# Autodesk Inventor assembly: Assembly
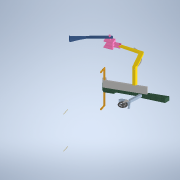
[picture p0: Inventor's stored thumbnail of the model, 180x180]
Saved by Autodesk Inventor 2021 (Build 250183000, 183)
## iProperties
Created: 2021-05-09
Part Number: Assembly
Document SubType Name: Assembly
Designer: Alsayaary
Author: Abdulrahman
## Documents named in this file (11)
- C:\Users\ocon0143\OneDrive - Flinders\Advn Mech Design Shared\6_Development\2_Design\inventor\securing_mechanism\Assembly.iam
- C:\Users\ocon0143\OneDrive - Flinders\Advn Mech Design Shared\6_Development\2_Design\inventor\securing_mechanism\grip - C1-1.ipt
- C:\Users\ocon0143\OneDrive - Flinders\Advn Mech Design Shared\6_Development\2_Design\inventor\securing_mechanism\grip - C2-1.ipt
- C:\Users\ocon0143\OneDrive - Flinders\Advn Mech Design Shared\6_Development\2_Design\inventor\securing_mechanism\grip - C4-1.ipt
- C:\Users\ocon0143\OneDrive - Flinders\Advn Mech Design Shared\6_Development\2_Design\inventor\securing_mechanism\pin-1.ipt
- C:\Users\ocon0143\OneDrive - Flinders\Advn Mech Design Shared\6_Development\2_Design\inventor\securing_mechanism\sweep.ipt
- C:\Users\ocon0143\OneDrive - Flinders\Advn Mech Design Shared\6_Development\2_Design\inventor\securing_mechanism\wheel2.ipt
- C:\Users\ocon0143\OneDrive - Flinders\Advn Mech Design Shared\6_Development\2_Design\inventor\securing_mechanism\grip - Copy1-1.ipt
- C:\Users\ocon0143\OneDrive - Flinders\Advn Mech Design Shared\6_Development\2_Design\inventor\securing_mechanism\handle.ipt
- C:\Users\ocon0143\OneDrive - Flinders\Advn Mech Design Shared\6_Development\2_Design\inventor\securing_mechanism\grip_N_fix.ipt
- C:\Users\ocon0143\OneDrive - Flinders\Advn Mech Design Shared\6_Development\2_Design\inventor\securing_mechanism\secure_wheel_bar.ipt
## Components (10 placed, 10 different names)
1. grip - C1-1:1 — Mate:1, Mate:2, Flush:1, Mate:3, Flush:2, Mate:4, Mate:5, Mate:7, Mate:8, Flush:3, Mate:14, Transitional:1, Mate:23
2. grip - C2-1:1 — Mate:5, Mate:7, Mate:8, Flush:3, Mate:16, Mate:17, Mate:19, Mate:22
3. grip - C4-1:1 — Mate:3, Flush:2, Mate:4, Mate:15
4. sweep:1 — Mate:9, Mate:10, Transitional:1
5. wheel2:1 — Mate:15, Angle:3
6. pin-1:2 — Mate:16, Mate:18
7. grip - Copy1-1:1 — Mate:17, Mate:18, Mate:19, Mate:20, Mate:21
8. handle:1 — Mate:20, Mate:21
9. grip_N_fix:1 — Mate:23
10. secure_wheel_bar:1 — Mate:22
## Relationships (30: Mate 21, Flush 4, Angle 3, Symmetry 1, Transitional 1)
- Mate:1: grip - C1-1:1
- Mate:2: grip - C1-1:1
- Flush:1: grip - C1-1:1
- Mate:3: grip - C1-1:1 ↔ grip - C4-1:1
- Flush:2 (6.27 mm): grip - C1-1:1 ↔ grip - C4-1:1
- Mate:4 (231.798 mm): grip - C1-1:1 ↔ grip - C4-1:1
- Mate:5: grip - C1-1:1 ↔ grip - C2-1:1
- Mate:7: grip - C1-1:1 ↔ grip - C2-1:1
- Mate:8 (313.691 mm): grip - C1-1:1 ↔ grip - C2-1:1
- Flush:3: grip - C1-1:1 ↔ grip - C2-1:1
- Mate:9: sweep:1
- Mate:10: sweep:1
- Mate:11
- Angle:1 (0 deg)
- Mate:12
- Angle:2 (0 deg)
- Symmetry:1
- Flush:4
- Mate:14: grip - C1-1:1
- Mate:15: grip - C4-1:1 ↔ wheel2:1
- Angle:3 (0 deg): wheel2:1
- Mate:16: grip - C2-1:1 ↔ pin-1:2
- Transitional:1: grip - C1-1:1 ↔ sweep:1
- Mate:17: grip - C2-1:1 ↔ grip - Copy1-1:1
- Mate:18: pin-1:2 ↔ grip - Copy1-1:1
- Mate:19 (2 mm): grip - C2-1:1 ↔ grip - Copy1-1:1
- Mate:20: grip - Copy1-1:1 ↔ handle:1
- Mate:21 (5 mm): grip - Copy1-1:1 ↔ handle:1
- Mate:22: grip - C2-1:1 ↔ secure_wheel_bar:1
- Mate:23: grip - C1-1:1 ↔ grip_N_fix:1
